# Autodesk Inventor assembly: CIMple Box
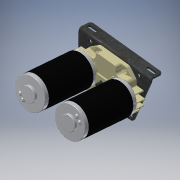
[picture p0: Inventor's stored thumbnail of the model, 180x180]
Saved by Autodesk Inventor 2016 (Build 200138000, 138)
## iProperties
Company: Unknown
Created: 2016-01-16
Part Number: CIMple Box
Description: Unknown
Document SubType Name: Assembly
Designer: gus
Mass: 2850.9 g
Surface Area: 1545.41 cm^2
Volume: 901.051 cm^3
Density: 3.16398 g/cm^3
User Status: complete
Sending System: Unknown
Preprocessor: XStep 1.0
Title: S:/Products/Gearboxes Spur Single Stage/Single Stage Toughbox/CIMple Box.stp
Author: Unknown
Revision Number: NONE
## Documents named in this file (12)
- \\Mac\Home\Desktop\1510-stronghold-CAD-master\chassis\CIMple Box\CIMple Box.iam
- \\Mac\Home\Desktop\1510-stronghold-CAD-master\chassis\CIMple Box\Single_d01.ipt
- \\Mac\Home\Desktop\1510-stronghold-CAD-master\chassis\CIMple Box\10-32x0625_shcs.ipt
- \\Mac\Home\Desktop\1510-stronghold-CAD-master\chassis\CIMple Box\r6zz.ipt
- \\Mac\Home\Desktop\1510-stronghold-CAD-master\chassis\CIMple Box\Single_d03.ipt
- \\Mac\Home\Desktop\1510-stronghold-CAD-master\chassis\CIMple Box\Single_d04.ipt
- \\Mac\Home\Desktop\1510-stronghold-CAD-master\chassis\CIMple Box\Single_d02.ipt
- \\Mac\Home\Desktop\1510-stronghold-CAD-master\chassis\CIMple Box\fr-8-zz.ipt
- \\Mac\Home\Desktop\1510-stronghold-CAD-master\chassis\CIMple Box\CIM motor.ipt
- \\Mac\Home\Desktop\1510-stronghold-CAD-master\chassis\CIMple Box\250_washer.ipt
- \\Mac\Home\Desktop\1510-stronghold-CAD-master\chassis\CIMple Box\14-20x0500_bhcs.ipt
- \\Mac\Home\Desktop\1510-stronghold-CAD-master\chassis\CIMple Box\Single_d05.ipt
## Components (16 placed, 11 different names)
1. Single_d01 — Rotational:1, Rotational:2, Rotational:3, Rotational:4, Rotational:5, Rotational:6, Mate:7, Mate:11
2. 10-32x0625_shcs — Rotational:2
3. 10-32x0625_shcs:5 — Rotational:1
4. 10-32x0625_shcs:6 — Rotational:3
5. 10-32x0625_shcs:7 — Rotational:4, Mate:6
6. r6zz — Cylindrical:1, Flush:2
7. Single_d03 — Cylindrical:1, Mate:1, Flush:1, Mate:2, Cylindrical:2, Flush:2, Rotational:7
8. Single_d04 — Mate:1, Flush:1, Mate:2, Mate:5
9. Single_d02 — Mate:8, Mate:9, Mate:10, Mate:11, Mate:12
10. fr-8-zz — Cylindrical:2, Mate:5, Mate:8, Mate:12
11. CIM motor — Cylindrical:3, Rotational:5, Rotational:6, Mate:10
12. CIM motor:1 — Cylindrical:4, Mate:6, Mate:7, Mate:9
13. 250_washer — Rotational:7, Rotational:8
14. 14-20x0500_bhcs — Rotational:8
15. Single_d05 — Cylindrical:3
16. Single_d05:1 — Cylindrical:4
## Relationships (24: Mate 10, RevoluteJoint 8, CylindricalJoint 4, Flush 2)
- Cylindrical:1: r6zz ↔ Single_d03
- Mate:1: Single_d03 ↔ Single_d04
- Flush:1: Single_d03 ↔ Single_d04
- Mate:2: Single_d03 ↔ Single_d04
- Cylindrical:2: Single_d03 ↔ fr-8-zz
- Flush:2: r6zz ↔ Single_d03
- Mate:5: Single_d04 ↔ fr-8-zz
- Cylindrical:3: CIM motor ↔ Single_d05
- Cylindrical:4: CIM motor:1 ↔ Single_d05:1
- Rotational:1 [RevoluteJoint]: Single_d01 ↔ 10-32x0625_shcs:5
- Rotational:2 [RevoluteJoint]: Single_d01 ↔ 10-32x0625_shcs
- Rotational:3 [RevoluteJoint]: Single_d01 ↔ 10-32x0625_shcs:6
- Rotational:4 [RevoluteJoint]: Single_d01 ↔ 10-32x0625_shcs:7
- Rotational:5 [RevoluteJoint]: Single_d01 ↔ CIM motor
- Rotational:6 [RevoluteJoint]: Single_d01 ↔ CIM motor
- Mate:6: 10-32x0625_shcs:7 ↔ CIM motor:1
- Mate:7: Single_d01 ↔ CIM motor:1
- Rotational:7 [RevoluteJoint]: Single_d03 ↔ 250_washer
- Rotational:8 [RevoluteJoint]: 250_washer ↔ 14-20x0500_bhcs
- Mate:8: Single_d02 ↔ fr-8-zz
- Mate:9: Single_d02 ↔ CIM motor:1
- Mate:10: Single_d02 ↔ CIM motor
- Mate:11: Single_d01 ↔ Single_d02
- Mate:12: Single_d02 ↔ fr-8-zz
